# Autodesk Inventor assembly: ARM_008_IntermediateBar
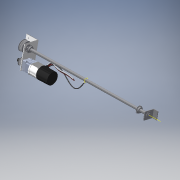
[picture p0: Inventor's stored thumbnail of the model, 180x180]
Saved by Autodesk Inventor 2018.3 (Build 223284000, 284)
## iProperties
Created: 2020-02-01
Part Number: ARM_008_IntermediateBar
Document SubType Name: Assembly
Designer: 21vogecale
Author: 21vogecale
## Documents named in this file (10)
- C:\Users\22barlalex\Documents\GrabCAD\Infinite Recharge 2020\Build season\ARM_008_IntermediateBar.iam
- C:\Users\22barlalex\Documents\GrabCAD\Infinite Recharge 2020\Build season\DGB STEP\217-4006_0_500_flanged_thunderhex_bearing.ipt
- C:\Users\22barlalex\Documents\GrabCAD\Infinite Recharge 2020\Build season\ARM_007_LongShaft.ipt
- C:\Users\22barlalex\Documents\GrabCAD\Infinite Recharge 2020\Build season\ARM_061__16t_Aluminum_Hub_Sprocket_25_Chain_1_2_Hex_Bore_217-2642.ipt
- C:\Users\22barlalex\Documents\GrabCAD\Infinite Recharge 2020\Brainstorming\Sam's Brainstorming Folder\Neo with versaplanetary two stage.iam
- C:\Users\22barlalex\Documents\GrabCAD\Infinite Recharge 2020\Build season\ARM_067_NewLongShaftMount.ipt
- C:\Users\22barlalex\Documents\GrabCAD\Infinite Recharge 2020\Build season\ARM_011_BearingMount.ipt
- C:\Users\22barlalex\Documents\GrabCAD\Infinite Recharge 2020\Build season\ARM_069_SDP_a_6a55m020df1506.ipt
- C:\Users\22barlalex\Documents\GrabCAD\Infinite Recharge 2020\Build season\ARM_070_SDP_a_6a55m030df1512.ipt
- C:\Users\22barlalex\Documents\GrabCAD\Infinite Recharge 2020\Build season\IntakeChain.ipt
## Components (12 placed, 9 different names)
1. 217-4006_0_500_flanged_thunderhex_bearing:1 — Flush:3, Mate:27, Mate:28, Mate:29, Mate:37
2. 217-4006_0_500_flanged_thunderhex_bearing:2 — Mate:19, Mate:21, Mate:24, Mate:26, Mate:33
3. ARM_007_LongShaft:1 — Mate:19, Flush:3, Mate:20, Angle:1, Mate:28, Angle:2, Mate:31, Angle:3, Flush:6, Flush:7, Mate:36
4. ARM_061__16t_Aluminum_Hub_Sprocket_25_Chain_1_2_Hex_Bore_217-2642:1 — Mate:20, Angle:1, Flush:8, Mate:39
5. ARM_061__16t_Aluminum_Hub_Sprocket_25_Chain_1_2_Hex_Bore_217-2642:2 — Mate:21, Flush:7, Flush:8, Mate:38
6. Neo with versaplanetary two stage:1 [sub-assembly] — Mate:32, Angle:4, Mate:34, Angle:5, Mate:35
7. ARM_067_NewLongShaftMount:1 — Mate:24, Mate:26, Angle:2, Mate:34, Angle:5, Angle:6, Mate:35
8. ARM_011_BearingMount:1 — Mate:27, Mate:29, Angle:6
9. ARM_069_SDP_a_6a55m020df1506:1 — Mate:32, Angle:4, Flush:5
10. ARM_070_SDP_a_6a55m030df1512:1 — Mate:31, Angle:3, Flush:5, Mate:33, Flush:6
11. IntakeChain:1 — Mate:36, Mate:38, Mate:40
12. IntakeChain:2 — Mate:37, Mate:39, Mate:40
## Relationships (29: Mate 18, Angle 6, Flush 5)
- Mate:19: 217-4006_0_500_flanged_thunderhex_bearing:2 ↔ ARM_007_LongShaft:1
- Flush:3 (-2.3368 mm): 217-4006_0_500_flanged_thunderhex_bearing:1 ↔ ARM_007_LongShaft:1
- Mate:20: ARM_007_LongShaft:1 ↔ ARM_061__16t_Aluminum_Hub_Sprocket_25_Chain_1_2_Hex_Bore_217-2642:1
- Angle:1 (0 deg): ARM_007_LongShaft:1 ↔ ARM_061__16t_Aluminum_Hub_Sprocket_25_Chain_1_2_Hex_Bore_217-2642:1
- Mate:21: 217-4006_0_500_flanged_thunderhex_bearing:2 ↔ ARM_061__16t_Aluminum_Hub_Sprocket_25_Chain_1_2_Hex_Bore_217-2642:2
- Mate:24: 217-4006_0_500_flanged_thunderhex_bearing:2 ↔ ARM_067_NewLongShaftMount:1
- Mate:26: 217-4006_0_500_flanged_thunderhex_bearing:2 ↔ ARM_067_NewLongShaftMount:1
- Mate:27: 217-4006_0_500_flanged_thunderhex_bearing:1 ↔ ARM_011_BearingMount:1
- Mate:28: 217-4006_0_500_flanged_thunderhex_bearing:1 ↔ ARM_007_LongShaft:1
- Mate:29: 217-4006_0_500_flanged_thunderhex_bearing:1 ↔ ARM_011_BearingMount:1
- Angle:2 (0 deg): ARM_007_LongShaft:1 ↔ ARM_067_NewLongShaftMount:1
- Mate:31: ARM_007_LongShaft:1 ↔ ARM_070_SDP_a_6a55m030df1512:1
- Angle:3 (0 deg): ARM_007_LongShaft:1 ↔ ARM_070_SDP_a_6a55m030df1512:1
- Mate:32: Neo with versaplanetary two stage:1 ↔ ARM_069_SDP_a_6a55m020df1506:1
- Angle:4 (0 deg): Neo with versaplanetary two stage:1 ↔ ARM_069_SDP_a_6a55m020df1506:1
- Flush:5: ARM_069_SDP_a_6a55m020df1506:1 ↔ ARM_070_SDP_a_6a55m030df1512:1
- Mate:33: 217-4006_0_500_flanged_thunderhex_bearing:2 ↔ ARM_070_SDP_a_6a55m030df1512:1
- Flush:6: ARM_007_LongShaft:1 ↔ ARM_070_SDP_a_6a55m030df1512:1
- Mate:34: Neo with versaplanetary two stage:1 ↔ ARM_067_NewLongShaftMount:1
- Angle:5 (90 deg): Neo with versaplanetary two stage:1 ↔ ARM_067_NewLongShaftMount:1
- Angle:6 (0 deg): ARM_067_NewLongShaftMount:1 ↔ ARM_011_BearingMount:1
- Flush:7 (38.0238 mm): ARM_007_LongShaft:1 ↔ ARM_061__16t_Aluminum_Hub_Sprocket_25_Chain_1_2_Hex_Bore_217-2642:2
- Flush:8 (-589.407 mm): ARM_061__16t_Aluminum_Hub_Sprocket_25_Chain_1_2_Hex_Bore_217-2642:1 ↔ ARM_061__16t_Aluminum_Hub_Sprocket_25_Chain_1_2_Hex_Bore_217-2642:2
- Mate:35: Neo with versaplanetary two stage:1 ↔ ARM_067_NewLongShaftMount:1
- Mate:36: ARM_007_LongShaft:1 ↔ IntakeChain:1
- Mate:37: 217-4006_0_500_flanged_thunderhex_bearing:1 ↔ IntakeChain:2
- Mate:38: ARM_061__16t_Aluminum_Hub_Sprocket_25_Chain_1_2_Hex_Bore_217-2642:2 ↔ IntakeChain:1
- Mate:39: ARM_061__16t_Aluminum_Hub_Sprocket_25_Chain_1_2_Hex_Bore_217-2642:1 ↔ IntakeChain:2
- Mate:40: IntakeChain:1 ↔ IntakeChain:2
